# Autodesk Inventor assembly: Custom_Delta_Assembly
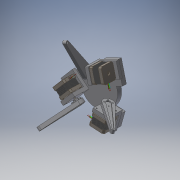
[picture p0: Inventor's stored thumbnail of the model, 180x180]
Saved by Autodesk Inventor 2019 (Build 230136000, 136)
## iProperties
Created: 2019-07-06
Part Number: Custom_Delta_Assembly
Document SubType Name: Assembly
Designer: Jorian Brusind
Author: Jorian Brusind
## Documents named in this file (6)
- C:\Users\Jorian Brusind\Documents\GitHub\ECE44x_Senior_Design\Design files\Delta Robot Arm\Inventor Files\Custom_Delta\Custom_Delta_Assembly.iam
- C:\Users\Jorian Brusind\Documents\GitHub\ECE44x_Senior_Design\Design files\Delta Robot Arm\Inventor Files\Custom_Delta\Stepper_Face.ipt
- C:\Users\Jorian Brusind\Documents\GitHub\ECE44x_Senior_Design\Design files\Delta Robot Arm\Inventor Files\nema-17-stepper-motor-with-v2-damper-1.snapshot.3\Nema 17  Stepper Motor length 34mm.ipt
- C:\Users\Jorian Brusind\Documents\GitHub\ECE44x_Senior_Design\Design files\Delta Robot Arm\Inventor Files\Stepper_Collar\products\12488\step\model.ipt
- C:\Users\Jorian Brusind\Documents\GitHub\ECE44x_Senior_Design\Design files\Delta Robot Arm\Inventor Files\Custom_Delta\Delta_Arm.ipt
- C:\Users\Jorian Brusind\Documents\GitHub\ECE44x_Senior_Design\Design files\Delta Robot Arm\Inventor Files\Custom_Delta\Delta_Top.ipt
## Components (13 placed, 5 different names)
1. Stepper_Face:1 — Mate:1, Mate:2, Mate:3, Mate:24, Mate:25, Mate:26
2. Nema 17  Stepper Motor length 34mm:1 — Mate:1, Mate:2, Mate:3, Mate:4, Flush:1
3. model:1 — Mate:4, Flush:1, Mate:7, Mate:8, Mate:9
4. Delta_Arm:1 — Mate:7, Mate:8, Flush:2, Mate:9
5. Stepper_Face:2 — Mate:32, Mate:33, Mate:34
6. Nema 17  Stepper Motor length 34mm:2
7. model:2
8. Delta_Arm:2
9. Stepper_Face:3 — Mate:27, Mate:28, Mate:29
10. Nema 17  Stepper Motor length 34mm:3
11. model:3
12. Delta_Arm:3
13. Delta_Top:1 — Mate:24, Mate:25, Mate:26, Mate:27, Mate:28, Mate:29, Mate:32, Mate:33, Mate:34
## Relationships (34: Mate 30, Flush 4)
- Mate:1: Stepper_Face:1 ↔ Nema 17  Stepper Motor length 34mm:1
- Mate:2: Stepper_Face:1 ↔ Nema 17  Stepper Motor length 34mm:1
- Mate:3: Stepper_Face:1 ↔ Nema 17  Stepper Motor length 34mm:1
- Mate:4: Nema 17  Stepper Motor length 34mm:1 ↔ model:1
- Flush:1: Nema 17  Stepper Motor length 34mm:1 ↔ model:1
- Mate:7: model:1 ↔ Delta_Arm:1
- Mate:8: model:1 ↔ Delta_Arm:1
- Flush:2: Delta_Arm:1
- Mate:9: model:1 ↔ Delta_Arm:1
- [Mate]: Stepper_Face:2 ↔ Nema 17  Stepper Motor length 34mm:2
- [Mate]: Stepper_Face:2 ↔ Nema 17  Stepper Motor length 34mm:2
- [Mate]: Stepper_Face:2 ↔ Nema 17  Stepper Motor length 34mm:2
- [Mate]: Nema 17  Stepper Motor length 34mm:2 ↔ model:2
- [Flush]: Nema 17  Stepper Motor length 34mm:2 ↔ model:2
- [Mate]: model:2 ↔ Delta_Arm:2
- [Mate]: model:2 ↔ Delta_Arm:2
- [Mate]: model:2 ↔ Delta_Arm:2
- [Mate]: Stepper_Face:3 ↔ Nema 17  Stepper Motor length 34mm:3
- [Mate]: Stepper_Face:3 ↔ Nema 17  Stepper Motor length 34mm:3
- [Mate]: Stepper_Face:3 ↔ Nema 17  Stepper Motor length 34mm:3
- [Mate]: Nema 17  Stepper Motor length 34mm:3 ↔ model:3
- [Flush]: Nema 17  Stepper Motor length 34mm:3 ↔ model:3
- [Mate]: model:3 ↔ Delta_Arm:3
- [Mate]: model:3 ↔ Delta_Arm:3
- [Mate]: model:3 ↔ Delta_Arm:3
- Mate:24: Stepper_Face:1 ↔ Delta_Top:1
- Mate:25: Stepper_Face:1 ↔ Delta_Top:1
- Mate:26: Stepper_Face:1 ↔ Delta_Top:1
- Mate:27: Stepper_Face:3 ↔ Delta_Top:1
- Mate:28: Stepper_Face:3 ↔ Delta_Top:1
- Mate:29: Stepper_Face:3 ↔ Delta_Top:1
- Mate:32: Stepper_Face:2 ↔ Delta_Top:1
- Mate:33: Stepper_Face:2 ↔ Delta_Top:1
- Mate:34: Stepper_Face:2 ↔ Delta_Top:1
## Named parameters: d13_d12 = 0 mm, d14_d5 = 0 mm, d15_d7 = 0 mm, d16_d8 = 0 mm, d17_d0 = 0 mm, d18_d1 = 0 mm, d19_d2 = 0 mm, d20_d3 = 0 mm, d21_d12 = 0 mm, d22_d5 = 0 mm, d23_d7 = 0 mm, d24_d8 = 0 mm, d25_d0 = 0 mm, d26_d1 = 0 mm, d27_d2 = 0 mm, d28_d3 = 0 mm
